# Autodesk Inventor assembly: 775pro_2_E_Female
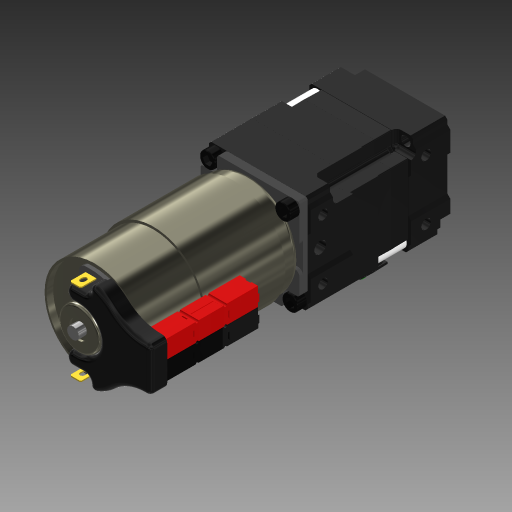
[picture p0: Inventor's stored thumbnail of the model, 512x512]
Saved by Autodesk Inventor 2023 (Build 270158000, 158)
## iProperties
Created: 2018-08-19
Part Number: 775pro_2_E_Female
Document SubType Name: Assembly
Mass: 1123.04 g
Surface Area: 1203.25 cm^2
Volume: 285.054 cm^3
Density: 3.93975 g/cm^3
## Documents named in this file (11)
- C:\Users\Cal\Desktop\Robotics\Design\Collaborative\Collaborative Parts Library\General Gearboxes\Planetaries\Versaplanetary\VersaPlanetary\775pro, 2 Stages, Encoder, Female Output.iam
- C:\Users\Cal\Desktop\Robotics\Design\Collaborative\Collaborative Parts Library\General Gearboxes\Planetaries\Versaplanetary\V2 Stages\V2 Output Stage.iam
- C:\Users\Cal\Desktop\Robotics\Design\Collaborative\Collaborative Parts Library\General Gearboxes\Planetaries\Versaplanetary\Intermediate Stages\Ring Gear.ipt
- C:\Users\Cal\Desktop\Robotics\Design\Collaborative\Collaborative Parts Library\General Gearboxes\Planetaries\Versaplanetary\Intermediate Stages\VP Encoder.iam
- C:\Users\Cal\Desktop\Robotics\Design\Collaborative\Collaborative Parts Library\General Gearboxes\Planetaries\Versaplanetary\V2 Stages\V2 Input Stage.iam
- C:\Users\Cal\Desktop\Robotics\Design\Collaborative\Collaborative Parts Library\General Gearboxes\Planetaries\Versaplanetary\Screws\8-32 x 2.25in Screw.ipt
- C:\Users\Cal\Desktop\Robotics\Design\Collaborative\Collaborative Parts Library\Power Transfer\Bearings and Bushings\Bearings\6902ZZ.ipt
- E:\Middleton Robotics\Collaborative Robots\Collaborative Part Library\Power Transfer\Bearings.ipt
- C:\Users\Cal\Desktop\Robotics\Design\Collaborative\Collaborative Parts Library\General Gearboxes\Planetaries\Versaplanetary\V2 Stages\V2 Input Stage\VP 775pro Input.iam
- C:\Users\Cal\Desktop\Robotics\Design\Collaborative\Collaborative Parts Library\General Gearboxes\Planetaries\Versaplanetary\V2 Stages\V2 Output Stage\VP V2 Output Stage Female.iam
- C:\Users\Cal\Desktop\Robotics\Design\Collaborative\Collaborative Parts Library\General Gearboxes\Planetaries\Versaplanetary\VersaPlanetary.iam
## Components (8 placed, 6 different names)
1. VP V2 Output Stage Female:3 [sub-assembly] — EncoderConstraint1, EncoderConstraint2, EncoderConstraint3, Flush:6, 2StageBasicInputMate2, Insert:25
2. Ring Gear 2 — Mate:4, Mate:5, Flush:6, 2StageBasicInputMate1
3. VP Encoder:1 [sub-assembly] — EncoderConstraint1, EncoderConstraint2, EncoderConstraint3, Mate:4, Mate:5
4. VP 775pro Input:1 [sub-assembly] — 2StageBasicInputMate1, 2StageBasicInputMate2, Insert:10, Insert:11
5. 8-32 x 2.25in Screw:1 — Insert:10
6. 8-32 x 2.25in Screw:2 — Insert:11
7. 6902ZZ:1
8. 6902ZZ:2 — Insert:25
## Relationships (11: Mate 4, Insert 4, Flush 2, Angle 1)
- EncoderConstraint1 [Mate]: VP V2 Output Stage Female:3 ↔ VP Encoder:1
- EncoderConstraint2 [Mate]: VP V2 Output Stage Female:3 ↔ VP Encoder:1
- EncoderConstraint3 [Angle] (0 deg): VP V2 Output Stage Female:3 ↔ VP Encoder:1
- Mate:4: Ring Gear 2 ↔ VP Encoder:1
- Mate:5: Ring Gear 2 ↔ VP Encoder:1
- Flush:6: VP V2 Output Stage Female:3 ↔ Ring Gear 2
- 2StageBasicInputMate1 [Insert]: Ring Gear 2 ↔ VP 775pro Input:1
- 2StageBasicInputMate2 [Flush]: VP V2 Output Stage Female:3 ↔ VP 775pro Input:1
- Insert:10: VP 775pro Input:1 ↔ 8-32 x 2.25in Screw:1
- Insert:11: VP 775pro Input:1 ↔ 8-32 x 2.25in Screw:2
- Insert:25: VP V2 Output Stage Female:3 ↔ 6902ZZ:2
